# Autodesk Inventor assembly: BevelGears
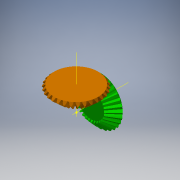
[picture p0: Inventor's stored thumbnail of the model, 180x180]
Saved by Autodesk Inventor 2017 (Build 210142000, 142)
## iProperties
Created: 2018-05-09
Part Number: BevelGears
Document SubType Name: Assembly
Designer: skhi8305
Author: skhi8305
## Documents named in this file (2)
- G:\FinalIEDProject\BevelGears.iam
- G:\FinalIEDProject\BevelGears\Design Accelerator\Bevel Gears1.iam
## Components (1 placed, 1 different names)
1. Bevel Gears:1 [sub-assembly] — Mate:1, Mate:2, Mate:3, Angle:1
## Relationships (4: Mate 3, Angle 1)
- Mate:1: Bevel Gears:1
- Mate:2: Bevel Gears:1
- Mate:3: Bevel Gears:1
- Angle:1 (360 deg): Bevel Gears:1
